# Autodesk Inventor assembly: forearm
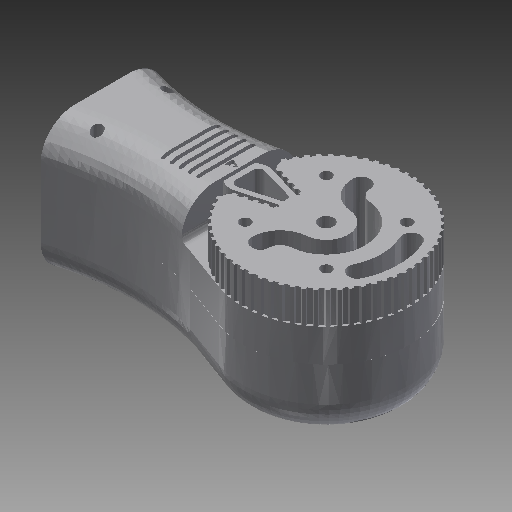
[picture p0: Inventor's stored thumbnail of the model, 512x512]
Saved by Autodesk Inventor 2019 (Build 230136000, 136)
## iProperties
Created: 2020-03-22
Part Number: forearm
Document SubType Name: Assembly
Designer: james
Author: james
## Documents named in this file (4)
- F:\JimsRobot\FIRSTRobots\Design\RBX1-REMIX\forearm\forearm.iam
- F:\JimsRobot\FIRSTRobots\Design\Library\McMaster\StepperMotor\Nema 17 6627T670_POSITION-CONTROL DC MOTOR.ipt
- F:\JimsRobot\FIRSTRobots\Design\RBX1-REMIX\forearm\forearm_left_qty1.ipt
- F:\JimsRobot\FIRSTRobots\Design\RBX1-REMIX\forearm\forearm_right_qty1.ipt
## Components (3 placed, 3 different names)
1. Nema 17 6627T670_POSITION-CONTROL DC MOTOR:1 — Mate:1, Mate:2
2. forearm_left_qty1:1 — Mate:3, Flush:1, Mate:4
3. forearm_right_qty1:1 — Mate:1, Mate:2, Mate:3, Flush:1, Mate:4
## Relationships (5: Mate 4, Flush 1)
- Mate:1: Nema 17 6627T670_POSITION-CONTROL DC MOTOR:1 ↔ forearm_right_qty1:1
- Mate:2: Nema 17 6627T670_POSITION-CONTROL DC MOTOR:1 ↔ forearm_right_qty1:1
- Mate:3: forearm_left_qty1:1 ↔ forearm_right_qty1:1
- Flush:1: forearm_left_qty1:1 ↔ forearm_right_qty1:1
- Mate:4: forearm_left_qty1:1 ↔ forearm_right_qty1:1
